# Autodesk Inventor assembly: z_assembly
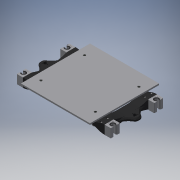
[picture p0: Inventor's stored thumbnail of the model, 180x180]
Saved by Autodesk Inventor 2017 (Build 210142000, 142)
## iProperties
Created: 2016-06-30
Part Number: z_assembly
Document SubType Name: Assembly
Designer: brent
Author: brent
## Documents named in this file (5)
- C:\Users\yibre\OneDrive\personal\printer_mechanical\z_assembly.iam
- C:\Users\yibre\OneDrive\personal\printer_mechanical\zaxis.ipt
- C:\Users\yibre\OneDrive\personal\printer_mechanical\offtheshelf\sbr12uu.ipt
- C:\Users\yibre\OneDrive\personal\printer_mechanical\z_assembly\Design Accelerator\Bolted Connection1.iam
- C:\Users\yibre\OneDrive\personal\printer_mechanical\z_assembly\Design Accelerator\Bolted Connection2.iam
## Components (25 placed, 3 different names)
1. zaxis:1 — Mate:9, Mate:10, Mate:11, Mate:12, Mate:13, Mate:14, Mate:15, Mate:16, Mate:17, Mate:18, Mate:19, Mate:20, Mate:21, Mate:22, Mate:23, Flush:1, Flush:2, Flush:3, Mate:24, Mate:25, Mate:26, Mate:27, Mate:28, Mate:29, Mate:30, Mate:31, Mate:32, Mate:33, Mate:34, Mate:35, Mate:36, Mate:37, Mate:38, Mate:39, Mate:40, Mate:41, Mate:42, Mate:43, Mate:44, Mate:45, Mate:46, Mate:47, Mate:48, Mate:49, Mate:50, Mate:51, Mate:52, Mate:53, Mate:54, Mate:55
2. sbr12uu:1 — Mate:17, Mate:18
3. sbr12uu:2 — Mate:14, Mate:15, Mate:16
4. sbr12uu:3 — Mate:11, Mate:12
5. sbr12uu:4 — Mate:9, Mate:10, Mate:13
6. Bolted Connection:1 [sub-assembly] — Mate:19, Mate:20
7. Bolted Connection:2 [sub-assembly] — Mate:21, Flush:3
8. Bolted Connection:3 [sub-assembly] — Mate:22, Flush:2
9. Bolted Connection:4 [sub-assembly] — Mate:23, Flush:1
10. Bolted Connection:5 [sub-assembly] — Mate:24, Mate:25
11. Bolted Connection:6 [sub-assembly] — Mate:29, Mate:39
12. Bolted Connection:7 [sub-assembly] — Mate:28, Mate:38
13. Bolted Connection:8 [sub-assembly] — Mate:32, Mate:35
14. Bolted Connection:9 [sub-assembly] — Mate:31, Mate:36
15. Bolted Connection:10 [sub-assembly] — Mate:33, Mate:34
16. Bolted Connection:11 [sub-assembly] — Mate:30, Mate:37
17. Bolted Connection:12 [sub-assembly] — Mate:26, Mate:27
18. Bolted Connection:13 [sub-assembly] — Mate:40, Mate:50
19. Bolted Connection:14 [sub-assembly] — Mate:41, Mate:51
20. Bolted Connection:15 [sub-assembly] — Mate:42, Mate:52
21. Bolted Connection:16 [sub-assembly] — Mate:47, Mate:48
22. Bolted Connection:17 [sub-assembly] — Mate:45, Mate:55
23. Bolted Connection:18 [sub-assembly] — Mate:46, Mate:49
24. Bolted Connection:19 [sub-assembly] — Mate:44, Mate:54
25. Bolted Connection:20 [sub-assembly] — Mate:43, Mate:53
## Relationships (50: Mate 47, Flush 3)
- Mate:9: zaxis:1 ↔ sbr12uu:4
- Mate:10: zaxis:1 ↔ sbr12uu:4
- Mate:11: zaxis:1 ↔ sbr12uu:3
- Mate:12: zaxis:1 ↔ sbr12uu:3
- Mate:13: zaxis:1 ↔ sbr12uu:4
- Mate:14: zaxis:1 ↔ sbr12uu:2
- Mate:15: zaxis:1 ↔ sbr12uu:2
- Mate:16: zaxis:1 ↔ sbr12uu:2
- Mate:17: zaxis:1 ↔ sbr12uu:1
- Mate:18: zaxis:1 ↔ sbr12uu:1
- Mate:19: zaxis:1 ↔ Bolted Connection:1
- Mate:20: zaxis:1 ↔ Bolted Connection:1
- Mate:21: zaxis:1 ↔ Bolted Connection:2
- Mate:22: zaxis:1 ↔ Bolted Connection:3
- Mate:23: zaxis:1 ↔ Bolted Connection:4
- Flush:1: zaxis:1 ↔ Bolted Connection:4
- Flush:2: zaxis:1 ↔ Bolted Connection:3
- Flush:3: zaxis:1 ↔ Bolted Connection:2
- Mate:24: zaxis:1 ↔ Bolted Connection:5
- Mate:25: zaxis:1 ↔ Bolted Connection:5
- Mate:26: zaxis:1 ↔ Bolted Connection:12
- Mate:27: zaxis:1 ↔ Bolted Connection:12
- Mate:28: zaxis:1 ↔ Bolted Connection:7
- Mate:29: zaxis:1 ↔ Bolted Connection:6
- Mate:30: zaxis:1 ↔ Bolted Connection:11
- Mate:31: zaxis:1 ↔ Bolted Connection:9
- Mate:32: zaxis:1 ↔ Bolted Connection:8
- Mate:33: zaxis:1 ↔ Bolted Connection:10
- Mate:34: zaxis:1 ↔ Bolted Connection:10
- Mate:35: zaxis:1 ↔ Bolted Connection:8
- Mate:36: zaxis:1 ↔ Bolted Connection:9
- Mate:37: zaxis:1 ↔ Bolted Connection:11
- Mate:38: zaxis:1 ↔ Bolted Connection:7
- Mate:39: zaxis:1 ↔ Bolted Connection:6
- Mate:40: zaxis:1 ↔ Bolted Connection:13
- Mate:41: zaxis:1 ↔ Bolted Connection:14
- Mate:42: zaxis:1 ↔ Bolted Connection:15
- Mate:43: zaxis:1 ↔ Bolted Connection:20
- Mate:44: zaxis:1 ↔ Bolted Connection:19
- Mate:45: zaxis:1 ↔ Bolted Connection:17
- Mate:46: zaxis:1 ↔ Bolted Connection:18
- Mate:47: zaxis:1 ↔ Bolted Connection:16
- Mate:48: zaxis:1 ↔ Bolted Connection:16
- Mate:49: zaxis:1 ↔ Bolted Connection:18
- Mate:50: zaxis:1 ↔ Bolted Connection:13
- Mate:51: zaxis:1 ↔ Bolted Connection:14
- Mate:52: zaxis:1 ↔ Bolted Connection:15
- Mate:53: zaxis:1 ↔ Bolted Connection:20
- Mate:54: zaxis:1 ↔ Bolted Connection:19
- Mate:55: zaxis:1 ↔ Bolted Connection:17
